# Autodesk Inventor assembly: Case
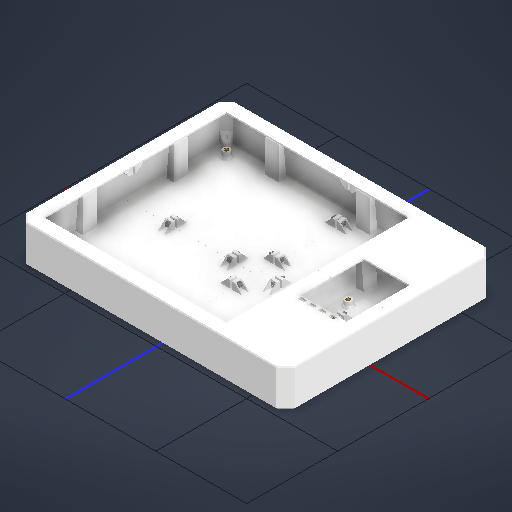
[picture p0: Inventor's stored thumbnail of the model, 512x512]
Saved by Autodesk Inventor 2026 (Build 300175000, 175)
## iProperties
Created: 2025-06-14
Part Number: Case
Document SubType Name: Assembly
Designer: ckyiu
Author: ckyiu
## Documents named in this file (4)
- F:\Chessboard-Design\Design\Case\Case.iam
- F:\Chessboard-Design\Design\Case\Bottom\Case Bottom.iam
- F:\Chessboard-Design\Design\Case\Top\Case Top.iam
- F:\Chessboard-Design\Design\Hardware\M2.5\Screws\(8mm) 92000A105_Passivated 18-8 Stainless Steel Pan Head Phillips Screws.ipt
## Components (6 placed, 3 different names)
1. Case Bottom:1 [sub-assembly] — Mate:1, Flush:1, Flush:2, Insert:1, Insert:2, Insert:3, Insert:4
2. Case Top:1 [sub-assembly] — Mate:1, Flush:1, Flush:2
3. (8mm) 92000A105_Passivated 18-8 Stainless Steel Pan Head Phillips Screws:1 — Insert:1
4. (8mm) 92000A105_Passivated 18-8 Stainless Steel Pan Head Phillips Screws:2 — Insert:2
5. (8mm) 92000A105_Passivated 18-8 Stainless Steel Pan Head Phillips Screws:3 — Insert:3
6. (8mm) 92000A105_Passivated 18-8 Stainless Steel Pan Head Phillips Screws:4 — Insert:4
## Relationships (7: Insert 4, Flush 2, Mate 1)
- Mate:1: Case Bottom:1 ↔ Case Top:1
- Flush:1: Case Bottom:1 ↔ Case Top:1
- Flush:2: Case Bottom:1 ↔ Case Top:1
- Insert:1: Case Bottom:1 ↔ (8mm) 92000A105_Passivated 18-8 Stainless Steel Pan Head Phillips Screws:1
- Insert:2: Case Bottom:1 ↔ (8mm) 92000A105_Passivated 18-8 Stainless Steel Pan Head Phillips Screws:2
- Insert:3: Case Bottom:1 ↔ (8mm) 92000A105_Passivated 18-8 Stainless Steel Pan Head Phillips Screws:3
- Insert:4: Case Bottom:1 ↔ (8mm) 92000A105_Passivated 18-8 Stainless Steel Pan Head Phillips Screws:4
